# Autodesk Inventor assembly: Application_Full-Fiedld_Time_Domain_OCT_combined_UC2-VCA
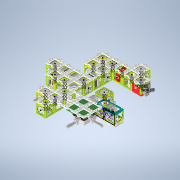
[picture p0: Inventor's stored thumbnail of the model, 180x180]
Saved by Autodesk Inventor 2022 (Build 260153000, 153)
## iProperties
Created: 2022-01-05
Part Number: Application_Full-Fiedld_Time_Domain_OCT_combined_UC2-VCA
Document SubType Name: Assembly
Designer: diederichbenedict
Author: diederichbenedict
## Documents named in this file (17)
- G:\My Drive\MODULE 4 - Master Thesis\2.Experiments\Modules\Application_Full-Field_Time_Domain_OCT_combined_UC2-VCA.iam
- G:\My Drive\MODULE 4 - Master Thesis\2.Experiments\Modules\7.Camera_Module\Assembly_Cube_AlliedVision_Alvium_v3.iam
- G:\My Drive\MODULE 4 - Master Thesis\2.Experiments\Modules\13.XY_Stage_with_Cubes\Assembly_XY_Linear_stage_with_Baseplates_v3.iam
- G:\My Drive\MODULE 4 - Master Thesis\2.Experiments\Modules\10.Lens_Thorlabs_Module\Assembly_Cube_Thorlabs_Lens_Cage_v3.iam
- G:\My Drive\MODULE 4 - Master Thesis\2.Experiments\Modules\1.Baseplate\Baseplate_IM\10_Base_puzzle_IM.ipt
- G:\My Drive\MODULE 4 - Master Thesis\2.Experiments\Modules\8.Beamsplitter_Module\Assembly_Cube_Beamsplitter_v3.iam
- G:\My Drive\MODULE 4 - Master Thesis\2.Experiments\Modules\14.Mirror_45_Kinematic_Module\Kinematic_Mirror_Holder_45_edge\Assembly_Cube_Kinematic_Mirrormount_Thorlabs_45_PRO_v3.iam
- G:\My Drive\MODULE 4 - Master Thesis\2.Experiments\Modules\12.Sample_Mirror_Module\Assembly_Cube_Kinematic_Mirrormount_Thorlabs_90_PRO_v3.iam
- G:\My Drive\MODULE 4 - Master Thesis\2.Experiments\Modules\14.Mirror_45_Kinematic_Module\Assembly_Cube_Kinematic_Mirrormount_45_base.iam
- G:\My Drive\MODULE 4 - Master Thesis\2.Experiments\Modules\4.SLD_Module\Assembly_Cube_SLD_Superlum_TO56_package.iam
- G:\My Drive\MODULE 4 - Master Thesis\2.Experiments\Modules\2.Base_Cube\Base_Cube_IM\Assembly_Cube_empty_IM_v3.iam
- G:\My Drive\MODULE 4 - Master Thesis\2.Experiments\Modules\6.Thorlabs_Pinhole\Assembly_Cube_Pinhole_v3.iam
- G:\My Drive\MODULE 4 - Master Thesis\2.Experiments\Modules\9.Adjustable_Z_Stage_Module\Manually_driven_MGN12H_Z_Stage\Assembly_Cube_Z-Stage_NEMA8_captive_v0.iam
- G:\My Drive\MODULE 4 - Master Thesis\2.Experiments\Modules\3.Laser_Module\Assembly_Cube_Laser_Multicolour_v3.iam
- G:\My Drive\MODULE 4 - Master Thesis\2.Experiments\Modules\11.Reference_Mirror_Module\Reference_Mirror_with_UC2-VCA_Module\Assembly_Cube_VCA_mirror.iam
- G:\My Drive\MODULE 4 - Master Thesis\2.Experiments\Modules\9.Adjustable_Z_Stage_Module\Manually_driven_MGN12H_XZ_Stage\Assembly_Cube_Z_Stage_Objective_XY_Stage_Module.iam
- G:\My Drive\MODULE 4 - Master Thesis\2.Experiments\Modules\9.Adjustable_Z_Stage_Module\Assembly_Cube_RMS_Objective_Holder_v3.iam
## Components (42 placed, 16 different names)
1. Assembly_Cube_Kinematic_Mirrormount_Thorlabs_90_PRO_v3:1 [sub-assembly] — Rigid:12
2. 10_Base_puzzle_IM:18 — Rigid:2, Rigid:43, Rigid:44
3. 10_Base_puzzle_IM:1 — Passend:1, Rigid:2, Rigid:3, Rigid:15
4. 10_Base_puzzle_IM:19 — Rigid:3, Rigid:4, Rigid:5, Rigid:6
5. 10_Base_puzzle_IM:21 — Rigid:6, Rigid:13, Rigid:20, Rigid:53
6. 10_Base_puzzle_IM:20 — Rigid:5, Rigid:7, Rigid:35
7. Assembly_Cube_AlliedVision_Alvium_v3:1 [sub-assembly] — Einfügen:4
8. 10_Base_puzzle_IM:17 — Einfügen:4, Rigid:14
9. Assembly_Cube_Beamsplitter_v3:1 [sub-assembly] — Rigid:4
10. 10_Base_puzzle_IM:22 — Rigid:7, Rigid:8, Rigid:10, Rigid:38
11. 10_Base_puzzle_IM:23 — Rigid:8, Rigid:12
12. 10_Base_puzzle_IM:25 — Rigid:10
13. 10_Base_puzzle_IM:24 — Rigid:11
14. Assembly_XY_Linear_stage_with_Baseplates_v3:1 [sub-assembly] — Rigid:11, Rigid:37, Rigid:40
15. 10_Base_puzzle_IM:27 — Rigid:14, Rigid:17, Rigid:42
16. 10_Base_puzzle_IM:26 — Rigid:13, Rigid:41
17. Assembly_Cube_Kinematic_Mirrormount_45_base:2 [sub-assembly] — Rigid:15
18. Assembly_Cube_Kinematic_Mirrormount_45_base:1 [sub-assembly] — Rigid:46
19. Assembly_Cube_Thorlabs_Lens_Cage_v3:2 [sub-assembly] — Rigid:42
20. 10_Base_puzzle_IM:28 — Rigid:17, Rigid:18
21. Assembly_Cube_SLD_Superlum_TO56_package:1 [sub-assembly] — Rigid:18
22. Assembly_Cube_empty_IM_v3:2 [sub-assembly] — Rigid:20
23. Assembly_Cube_Thorlabs_Lens_Cage_v3:1 [sub-assembly] — Rigid:29
24. Assembly_Cube_Kinematic_Mirrormount_Thorlabs_45_PRO_v3:1 [sub-assembly] — Rigid:45
25. Assembly_Cube_Kinematic_Mirrormount_Thorlabs_45_PRO_v3:2 [sub-assembly] — Rigid:49
26. 10_Base_puzzle_IM:32 — Rigid:29, Rigid:47, Rigid:48, Rigid:50
27. 10_Base_puzzle_IM:33 — Rigid:31, Rigid:32, Rigid:33, Rigid:52
28. Assembly_Cube_Pinhole_v3:1 [sub-assembly] — Rigid:51
29. Assembly_Cube_Z-Stage_NEMA8_captive_v0:1 [sub-assembly] — Rigid:31
30. 10_Base_puzzle_IM:34 — Rigid:32
31. Assembly_Cube_Laser_Multicolour_v3:1 [sub-assembly] — Rigid:33
32. Assembly_Cube_VCA_mirror:1 [sub-assembly] — Rigid:37
33. Assembly_Cube_empty_IM_v3:4 [sub-assembly] — Rigid:35
34. Assembly_Cube_Z-Stage_NEMA8_captive_v0:2 [sub-assembly] — Rigid:39
35. 10_Base_puzzle_IM:35 — Rigid:38, Rigid:39
36. Assembly_Cube_Z_Stage_Objective_XY_Stage_Module:1 [sub-assembly] — Rigid:40
37. Assembly_Cube_Thorlabs_Lens_Cage_v3:3 [sub-assembly] — Rigid:41
38. Assembly_Cube_Thorlabs_Lens_Cage_v3:4 [sub-assembly] — Rigid:43
39. 10_Base_puzzle_IM:36 — Rigid:44, Rigid:45, Rigid:46, Rigid:47
40. 10_Base_puzzle_IM:37 — Rigid:48, Rigid:49
41. 10_Base_puzzle_IM:38 — Rigid:50, Rigid:51, Rigid:52
42. Assembly_Cube_RMS_Objective_Holder_v3:1 [sub-assembly] — Rigid:53
## Relationships (41: WeldJoint 39, Mate 1, Insert 1)
- Passend:1 [Mate]: 10_Base_puzzle_IM:1
- Einfügen:4 [Insert]: Assembly_Cube_AlliedVision_Alvium_v3:1 ↔ 10_Base_puzzle_IM:17
- Rigid:2 [WeldJoint]: 10_Base_puzzle_IM:18 ↔ 10_Base_puzzle_IM:1
- Rigid:3 [WeldJoint]: 10_Base_puzzle_IM:1 ↔ 10_Base_puzzle_IM:19
- Rigid:4 [WeldJoint]: 10_Base_puzzle_IM:19 ↔ Assembly_Cube_Beamsplitter_v3:1
- Rigid:5 [WeldJoint]: 10_Base_puzzle_IM:19 ↔ 10_Base_puzzle_IM:20
- Rigid:6 [WeldJoint]: 10_Base_puzzle_IM:19 ↔ 10_Base_puzzle_IM:21
- Rigid:7 [WeldJoint]: 10_Base_puzzle_IM:20 ↔ 10_Base_puzzle_IM:22
- Rigid:8 [WeldJoint]: 10_Base_puzzle_IM:22 ↔ 10_Base_puzzle_IM:23
- [WeldJoint]: 10_Base_puzzle_IM:25 ↔ 10_Base_puzzle_IM:24
- Rigid:10 [WeldJoint]: 10_Base_puzzle_IM:22 ↔ 10_Base_puzzle_IM:25
- Rigid:11 [WeldJoint]: 10_Base_puzzle_IM:24 ↔ Assembly_XY_Linear_stage_with_Baseplates_v3:1
- Rigid:12 [WeldJoint]: Assembly_Cube_Kinematic_Mirrormount_Thorlabs_90_PRO_v3:1 ↔ 10_Base_puzzle_IM:23
- Rigid:13 [WeldJoint]: 10_Base_puzzle_IM:21 ↔ 10_Base_puzzle_IM:26
- Rigid:14 [WeldJoint]: 10_Base_puzzle_IM:17 ↔ 10_Base_puzzle_IM:27
- Rigid:15 [WeldJoint]: 10_Base_puzzle_IM:1 ↔ Assembly_Cube_Kinematic_Mirrormount_45_base:2
- Rigid:17 [WeldJoint]: 10_Base_puzzle_IM:27 ↔ 10_Base_puzzle_IM:28
- Rigid:18 [WeldJoint]: 10_Base_puzzle_IM:28 ↔ Assembly_Cube_SLD_Superlum_TO56_package:1
- Rigid:20 [WeldJoint]: 10_Base_puzzle_IM:21 ↔ Assembly_Cube_empty_IM_v3:2
- Rigid:29 [WeldJoint]: Assembly_Cube_Thorlabs_Lens_Cage_v3:1 ↔ 10_Base_puzzle_IM:32
- Rigid:31 [WeldJoint]: 10_Base_puzzle_IM:33 ↔ Assembly_Cube_Z-Stage_NEMA8_captive_v0:1
- Rigid:32 [WeldJoint]: 10_Base_puzzle_IM:33 ↔ 10_Base_puzzle_IM:34
- Rigid:33 [WeldJoint]: 10_Base_puzzle_IM:33 ↔ Assembly_Cube_Laser_Multicolour_v3:1
- Rigid:35 [WeldJoint]: 10_Base_puzzle_IM:20 ↔ Assembly_Cube_empty_IM_v3:4
- Rigid:37 [WeldJoint]: Assembly_XY_Linear_stage_with_Baseplates_v3:1 ↔ Assembly_Cube_VCA_mirror:1
- Rigid:38 [WeldJoint]: 10_Base_puzzle_IM:22 ↔ 10_Base_puzzle_IM:35
- Rigid:39 [WeldJoint]: Assembly_Cube_Z-Stage_NEMA8_captive_v0:2 ↔ 10_Base_puzzle_IM:35
- Rigid:40 [WeldJoint]: Assembly_XY_Linear_stage_with_Baseplates_v3:1 ↔ Assembly_Cube_Z_Stage_Objective_XY_Stage_Module:1
- Rigid:41 [WeldJoint]: 10_Base_puzzle_IM:26 ↔ Assembly_Cube_Thorlabs_Lens_Cage_v3:3
- Rigid:42 [WeldJoint]: 10_Base_puzzle_IM:27 ↔ Assembly_Cube_Thorlabs_Lens_Cage_v3:2
- Rigid:43 [WeldJoint]: 10_Base_puzzle_IM:18 ↔ Assembly_Cube_Thorlabs_Lens_Cage_v3:4
- Rigid:44 [WeldJoint]: 10_Base_puzzle_IM:18 ↔ 10_Base_puzzle_IM:36
- Rigid:45 [WeldJoint]: Assembly_Cube_Kinematic_Mirrormount_Thorlabs_45_PRO_v3:1 ↔ 10_Base_puzzle_IM:36
- Rigid:46 [WeldJoint]: Assembly_Cube_Kinematic_Mirrormount_45_base:1 ↔ 10_Base_puzzle_IM:36
- Rigid:47 [WeldJoint]: 10_Base_puzzle_IM:32 ↔ 10_Base_puzzle_IM:36
- Rigid:48 [WeldJoint]: 10_Base_puzzle_IM:32 ↔ 10_Base_puzzle_IM:37
- Rigid:49 [WeldJoint]: Assembly_Cube_Kinematic_Mirrormount_Thorlabs_45_PRO_v3:2 ↔ 10_Base_puzzle_IM:37
- Rigid:50 [WeldJoint]: 10_Base_puzzle_IM:32 ↔ 10_Base_puzzle_IM:38
- Rigid:51 [WeldJoint]: Assembly_Cube_Pinhole_v3:1 ↔ 10_Base_puzzle_IM:38
- Rigid:52 [WeldJoint]: 10_Base_puzzle_IM:33 ↔ 10_Base_puzzle_IM:38
- Rigid:53 [WeldJoint]: 10_Base_puzzle_IM:21 ↔ Assembly_Cube_RMS_Objective_Holder_v3:1
## Named parameters: d42_d40 = 0 mm
